# Autodesk Inventor assembly: SanladererBowdenExtruder
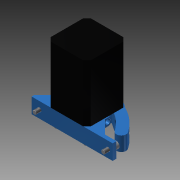
[picture p0: Inventor's stored thumbnail of the model, 180x180]
Saved by Autodesk Inventor 2015 SP1 (Build 190203100, 203)
## iProperties
Created: 2015-01-11
Part Number: SanladererBowdenExtruder
Document SubType Name: Assembly
Designer: Jack
Mass: 146.796 g
Surface Area: 300.5 cm^2
Volume: 137.998 cm^3
Density: 1.06375 g/cm^3
Author: Jack
Title: Sanladerer Bowden Extruder
## Documents named in this file (11)
- C:\Users\Jack\ownCloud\Projects\CoreXY\InventorModel\Extruder\SanladererBowdenExtruder\SanladererBowdenExtruder.iam
- C:\Users\Jack\ownCloud\Projects\CoreXY\InventorModel\Extruder\SanladererBowdenExtruder\SanladererBowdenArm.ipt
- C:\Users\Jack\ownCloud\Projects\CoreXY\InventorModel\Extruder\SanladererBowdenExtruder\SanladererBowdenBody.ipt
- C:\Users\Jack\ownCloud\Projects\CoreXY\InventorModel\Electronics\Motors\StepperMotorNema17.ipt
- C:\Users\Jack\ownCloud\Projects\CoreXY\InventorModel\Hardware\Extruder\DriveGearMK8.ipt
- C:\Users\Jack\ownCloud\Projects\CoreXY\InventorModel\Hardware\Bearing\BearingRadialBall\BearingRadialBall624zz.ipt
- C:\Users\Jack\ownCloud\Projects\CoreXY\InventorModel\Hardware\Bolts\SHCS\SHCS3\SHCS3x18.ipt
- C:\Users\Jack\ownCloud\Projects\CoreXY\InventorModel\Hardware\Wahsers\M3Washer.ipt
- C:\Users\Jack\ownCloud\Projects\CoreXY\InventorModel\Hardware\Bolts\SHCS\SHCS4\SHCS4x18.ipt
- C:\Users\Jack\ownCloud\Projects\CoreXY\InventorModel\Hardware\Wahsers\M4Washer.ipt
- C:\Users\Jack\ownCloud\Projects\CoreXY\InventorModel\Hardware\Bolts\SHCS\SHCS4\SHCS4x10.ipt
## Components (19 placed, 10 different names)
1. SanladererBowdenArm:1 — Mate:8, Mate:12, Mate:13, Mate:14, Mate:26, Mate:27, Mate:33, Mate:34
2. SanladererBowdenBody:1 — Mate:5, Mate:6, Mate:7, Mate:23, Mate:24, Mate:25, Mate:28, Mate:29, Mate:30, Mate:39, Mate:40, Mate:41, Mate:42
3. StepperMotorNema17:1 — Mate:5, Mate:6, Mate:7, Mate:8, Mate:10, Mate:11, Mate:12
4. DriveGearMK8:1 — Mate:10, Mate:11
5. BearingRadialBall624zz:1 — Mate:13, Mate:14
6. SHCS3x18:1 — Mate:18, Mate:19, Mate:23
7. SHCS3x18:2 — Mate:17, Mate:20, Mate:24
8. SHCS3x18:3 — Mate:16, Mate:21, Mate:25
9. SHCS3x18:4 — Mate:15, Mate:22, Mate:26
10. M3Washer:1 — Mate:18, Mate:19, Mate:28
11. M3Washer:2 — Mate:17, Mate:20, Mate:29
12. M3Washer:3 — Mate:16, Mate:21, Mate:30
13. M3Washer:4 — Mate:15, Mate:22, Mate:27
14. SHCS4x18:1 — Mate:31, Mate:32, Mate:33
15. M4Washer:1 — Mate:31, Mate:32, Mate:34
16. SHCS4x10:1 — Mate:36, Mate:37, Mate:40
17. SHCS4x10:2 — Mate:35, Mate:38, Mate:39
18. M4Washer:2 — Mate:35, Mate:38, Mate:42
19. M4Washer:3 — Mate:36, Mate:37, Mate:41
## Relationships (37: Mate 37)
- Mate:5: SanladererBowdenBody:1 ↔ StepperMotorNema17:1
- Mate:6: SanladererBowdenBody:1 ↔ StepperMotorNema17:1
- Mate:7: SanladererBowdenBody:1 ↔ StepperMotorNema17:1
- Mate:8: SanladererBowdenArm:1 ↔ StepperMotorNema17:1
- Mate:10: StepperMotorNema17:1 ↔ DriveGearMK8:1
- Mate:11 (3 mm): StepperMotorNema17:1 ↔ DriveGearMK8:1
- Mate:12: SanladererBowdenArm:1 ↔ StepperMotorNema17:1
- Mate:13: SanladererBowdenArm:1 ↔ BearingRadialBall624zz:1
- Mate:14: SanladererBowdenArm:1 ↔ BearingRadialBall624zz:1
- Mate:15: SHCS3x18:4 ↔ M3Washer:4
- Mate:16: SHCS3x18:3 ↔ M3Washer:3
- Mate:17: SHCS3x18:2 ↔ M3Washer:2
- Mate:18: SHCS3x18:1 ↔ M3Washer:1
- Mate:19: SHCS3x18:1 ↔ M3Washer:1
- Mate:20: SHCS3x18:2 ↔ M3Washer:2
- Mate:21: SHCS3x18:3 ↔ M3Washer:3
- Mate:22: SHCS3x18:4 ↔ M3Washer:4
- Mate:23: SanladererBowdenBody:1 ↔ SHCS3x18:1
- Mate:24: SanladererBowdenBody:1 ↔ SHCS3x18:2
- Mate:25: SanladererBowdenBody:1 ↔ SHCS3x18:3
- Mate:26: SanladererBowdenArm:1 ↔ SHCS3x18:4
- Mate:27: SanladererBowdenArm:1 ↔ M3Washer:4
- Mate:28: SanladererBowdenBody:1 ↔ M3Washer:1
- Mate:29: SanladererBowdenBody:1 ↔ M3Washer:2
- Mate:30: SanladererBowdenBody:1 ↔ M3Washer:3
- Mate:31: SHCS4x18:1 ↔ M4Washer:1
- Mate:32: SHCS4x18:1 ↔ M4Washer:1
- Mate:33: SanladererBowdenArm:1 ↔ SHCS4x18:1
- Mate:34: SanladererBowdenArm:1 ↔ M4Washer:1
- Mate:35: SHCS4x10:2 ↔ M4Washer:2
- Mate:36: SHCS4x10:1 ↔ M4Washer:3
- Mate:37: SHCS4x10:1 ↔ M4Washer:3
- Mate:38: SHCS4x10:2 ↔ M4Washer:2
- Mate:39: SanladererBowdenBody:1 ↔ SHCS4x10:2
- Mate:40: SanladererBowdenBody:1 ↔ SHCS4x10:1
- Mate:41: SanladererBowdenBody:1 ↔ M4Washer:3
- Mate:42: SanladererBowdenBody:1 ↔ M4Washer:2
